# Autodesk Inventor assembly: ЛЦМК.30000.20.00.00 СБ Держатель OLED
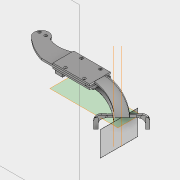
[picture p0: Inventor's stored thumbnail of the model, 180x180]
Saved by Autodesk Inventor 2021.2 (Build 252289000, 289)
## iProperties
Created: 2025-11-22
Part Number: ЛЦМК.30000.20.00.00 СБ Держатель OLED
Document SubType Name: Assembly
Designer: Захаров
Author: Захаров
## Documents named in this file (4)
- C:\Users\User\Documents\CaseARHead1\ЛЦМК.30000.20.00.00 Держатель OLED\ЛЦМК.30000.20.00.00 СБ Держатель OLED.iam
- C:\Users\User\Documents\CaseARHead1\ЛЦМК.30000.20.00.00 Держатель OLED\ЛЦМК.30000.20.00.01 Дужка.ipt
- C:\Users\User\Documents\CaseARHead1\ЛЦМК.30000.20.00.00 Держатель OLED\ЛЦМК.30000.20.00.02 Держатель OLED.ipt
- C:\Users\User\Documents\CaseARHead1\ЛЦМК.30000.20.00.00 Держатель OLED\OLED.ipt
## Components (3 placed, 3 different names)
1. ЛЦМК.30000.20.00.01 Дужка:1 — Вставка:1, Вставка:2, Вставка:3, Вставка:4
2. ЛЦМК.30000.20.00.02 Держатель OLED:1 — Вставка:1, Вставка:2
3. OLED:1 — Вставка:3, Вставка:4
## Relationships (4: Insert 4)
- Вставка:1 [Insert]: ЛЦМК.30000.20.00.01 Дужка:1 ↔ ЛЦМК.30000.20.00.02 Держатель OLED:1
- Вставка:2 [Insert]: ЛЦМК.30000.20.00.01 Дужка:1 ↔ ЛЦМК.30000.20.00.02 Держатель OLED:1
- Вставка:3 [Insert]: ЛЦМК.30000.20.00.01 Дужка:1 ↔ OLED:1
- Вставка:4 [Insert]: ЛЦМК.30000.20.00.01 Дужка:1 ↔ OLED:1
